# Autodesk Inventor assembly: AM-2235
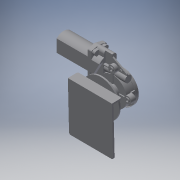
[picture p0: Inventor's stored thumbnail of the model, 180x180]
Saved by Autodesk Inventor 2016 SP1 (Build 200210100, 210)
## iProperties
Created: 2012-12-12
Part Number: AM-2235
Description: STEP AP203
Document SubType Name: Assembly
Designer: bbier
Sending System: SolidWorks 2010
Preprocessor: SwSTEP 2.0
Title: AM-2235.STEP
Revision Number: ANY
## Documents named in this file (9)
- C:\snobotics\CAD-Development\robSteele\SnoBotics2016\Brian Bierman\2015-02-05\x\AM-2235.iam
- C:\snobotics\CAD-Development\robSteele\SnoBotics2016\Brian Bierman\2015-02-05\x\AM-2235 output shaft.ipt
- C:\snobotics\CAD-Development\robSteele\SnoBotics2016\Brian Bierman\2015-02-05\x\AM-2235 gearbox housing.ipt
- C:\snobotics\CAD-Development\robSteele\SnoBotics2016\Brian Bierman\2015-02-05\x\AM-2235 threaded insert.ipt
- C:\snobotics\CAD-Development\robSteele\SnoBotics2016\Brian Bierman\2015-02-05\x\AM-2235 motor.ipt
- C:\snobotics\CAD-Development\robSteele\SnoBotics2016\Brian Bierman\2015-02-05\x\AM-2235 gear cap.ipt
- C:\snobotics\CAD-Development\robSteele\SnoBotics2016\Brian Bierman\2015-02-05\x\am-2279+10mm+DD+Bore+Hub.ipt
- C:\snobotics\CAD-Development\robSteele\SnoBotics2016\Brian Bierman\2015-02-05\x\sprocket.ipt
- C:\snobotics\CAD-Development\robSteele\SnoBotics2016\Brian Bierman\2015-02-05\x\snoBlowerBracket.ipt
## Components (10 placed, 10 different names)
1. AM-2235 output shaft_1 — Mate:2, Flush:1
2. AM-2235 gearbox housing_2
3. AM-2235 threaded insert_3
4. AM-2235 motor_4
5. AM-2235 threaded insert_5
6. AM-2235 threaded insert_6
7. AM-2235 gear cap_7
8. am-2279+10mm+DD+Bore+Hub:1 — Mate:2, Flush:1, Mate:3, Mate:4
9. sprocket:1 — Mate:3, Mate:4
10. snoBlowerBracket:1
## Relationships (4: Mate 3, Flush 1)
- Mate:2: AM-2235 output shaft_1 ↔ am-2279+10mm+DD+Bore+Hub:1
- Flush:1: AM-2235 output shaft_1 ↔ am-2279+10mm+DD+Bore+Hub:1
- Mate:3: am-2279+10mm+DD+Bore+Hub:1 ↔ sprocket:1
- Mate:4: am-2279+10mm+DD+Bore+Hub:1 ↔ sprocket:1
